# Autodesk Inventor assembly: 0deg
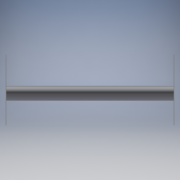
[picture p0: Inventor's stored thumbnail of the model, 180x180]
Saved by Autodesk Inventor 2018.2 (Build 222227000, 227)
## iProperties
Created: 2018-02-23
Part Number: 0deg
Material: 一般
Document SubType Name: Assembly
Designer: ku_sk
Author: ku_sk
## Documents named in this file (3)
- C:\Users\ku_sk\Documents\Inventor\AeroCAD2018\CAD\Inventor\Aero Parts\R-wing\type7-naca97\解析用\0deg.iam
- C:\Users\ku_sk\Documents\Inventor\AeroCAD2018\CAD\Inventor\Aero Parts\R-wing\type7-naca97\frap.ipt
- C:\Users\ku_sk\Documents\Inventor\AeroCAD2018\CAD\Inventor\Aero Parts\R-wing\type7-naca97\endplate.ipt
## Components (3 placed, 2 different names)
1. frap:1 — メイト:1, フラッシュ:1, メイト:2, メイト:3, メイト:4, メイト:5, 角度:2
2. endplate:1 — メイト:3, メイト:5, フラッシュ:2, フラッシュ:3
3. endplate:2 — メイト:2, メイト:4, フラッシュ:2, フラッシュ:3, 角度:1
## Relationships (10: Mate 5, Flush 3, Angle 2)
- メイト:1 [Mate]: frap:1
- フラッシュ:1 [Flush]: frap:1
- メイト:2 [Mate]: frap:1 ↔ endplate:2
- メイト:3 [Mate]: frap:1 ↔ endplate:1
- メイト:4 [Mate]: frap:1 ↔ endplate:2
- メイト:5 [Mate]: frap:1 ↔ endplate:1
- フラッシュ:2 [Flush]: endplate:1 ↔ endplate:2
- フラッシュ:3 [Flush]: endplate:1 ↔ endplate:2
- 角度:1 [Angle] (0 deg): endplate:2
- 角度:2 [Angle] (0 deg): frap:1
